# Autodesk Inventor assembly: правый привод_MIR1
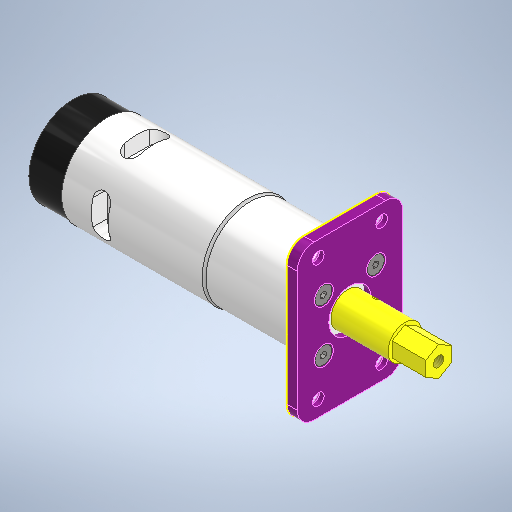
[picture p0: Inventor's stored thumbnail of the model, 512x512]
Saved by Autodesk Inventor 2025 (Build 290162000, 162)
## iProperties
Created: 2025-02-16
Part Number: правый привод_MIR1
Document SubType Name: Assembly
Designer: volko
Author: volko
## Documents named in this file (6)
- C:\Users\volko\Desktop\диплом\Модели\детали\правый привод_MIR1.iam
- C:\Users\volko\Desktop\диплом\Модели\Mecanum wheel - right\Mecanum wheel - right_MIR1.iam
- C:\Users\volko\Desktop\диплом\Модели\детали\CHP-42GP-775 ABHL_MIR2.ipt
- C:\Users\volko\Desktop\диплом\Модели\детали\кронштейн_MIR2.ipt
- C:\Users\volko\Desktop\диплом\Модели\детали\переходная втулка_MIR2.ipt
- C:\Users\volko\Desktop\диплом\Модели\детали\стандартные изделия\ru-RU\DIN 7991(2)\DIN 7991 - M4x8.ipt
## Components (8 placed, 5 different names)
1. Mecanum wheel - right_MIR1:1 [sub-assembly] — Совмещение:12, Совмещение:10, Совмещение:9, Совмещение:8
2. CHP-42GP-775 ABHL_MIR2:1 — Заподлицо:1, Совмещение:2, Совмещение:1, Совмещение:11, Совмещение:5, Совмещение:3, Совмещение:7, Совмещение:6
3. кронштейн_MIR2:1 — Совмещение:11, Совмещение:5, Совмещение:3, Совмещение:12, Совмещение:13, Совмещение:14, Совмещение:15
4. переходная втулка_MIR2:1 — Совмещение:10, Совмещение:9, Совмещение:8, Совмещение:7, Совмещение:6
5. DIN 7991 M4x8:1 — Совмещение:12
6. DIN 7991 M4x8:2 — Совмещение:13
7. DIN 7991 M4x8:3 — Совмещение:14
8. DIN 7991 M4x8:4 — Совмещение:15
## Relationships (16: Mate 15, Flush 1)
- Совмещение:12 [Mate]: Mecanum wheel - right_MIR1:1
- Заподлицо:1 [Flush]: CHP-42GP-775 ABHL_MIR2:1
- Совмещение:2 [Mate]: CHP-42GP-775 ABHL_MIR2:1
- Совмещение:1 [Mate]: CHP-42GP-775 ABHL_MIR2:1
- Совмещение:11 [Mate]: CHP-42GP-775 ABHL_MIR2:1 ↔ кронштейн_MIR2:1
- Совмещение:5 [Mate]: CHP-42GP-775 ABHL_MIR2:1 ↔ кронштейн_MIR2:1
- Совмещение:3 [Mate]: CHP-42GP-775 ABHL_MIR2:1 ↔ кронштейн_MIR2:1
- Совмещение:10 [Mate]: Mecanum wheel - right_MIR1:1 ↔ переходная втулка_MIR2:1
- Совмещение:9 [Mate]: Mecanum wheel - right_MIR1:1 ↔ переходная втулка_MIR2:1
- Совмещение:8 [Mate]: Mecanum wheel - right_MIR1:1 ↔ переходная втулка_MIR2:1
- Совмещение:7 [Mate]: CHP-42GP-775 ABHL_MIR2:1 ↔ переходная втулка_MIR2:1
- Совмещение:6 [Mate]: CHP-42GP-775 ABHL_MIR2:1 ↔ переходная втулка_MIR2:1
- Совмещение:12 [Mate]: кронштейн_MIR2:1 ↔ DIN 7991 M4x8:1
- Совмещение:13 [Mate]: кронштейн_MIR2:1 ↔ DIN 7991 M4x8:2
- Совмещение:14 [Mate]: кронштейн_MIR2:1 ↔ DIN 7991 M4x8:3
- Совмещение:15 [Mate]: кронштейн_MIR2:1 ↔ DIN 7991 M4x8:4
